# Autodesk Inventor assembly: Wheel Insert Inner Context
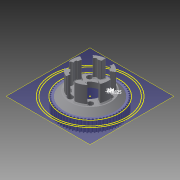
[picture p0: Inventor's stored thumbnail of the model, 180x180]
Saved by Autodesk Inventor 2015 SP1 (Build 190203100, 203)
## iProperties
Created: 2014-05-22
Part Number: Wheel Insert Inner Context
Document SubType Name: Assembly
Designer: dliu
Author: dliu
## Documents named in this file (3)
- C:\Users\dliu\Dropbox\dbhome\electric-longboard\dliu\Wheel Insert V3\Wheel Insert Inner V3 Context.iam
- C:\Users\dliu\Dropbox\dbhome\electric-longboard\dliu\Wheel Insert V3\Wheel Insert Sketch V3.ipt
- C:\Users\dliu\Dropbox\dbhome\electric-longboard\dliu\Wheel Insert V3\Wheel Insert Inner V3.ipt
## Components (2 placed, 2 different names)
1. Wheel Insert Sketch V3:1 — Mate:2, Mate:4, Mate:5
2. Wheel Insert Inner V3:1 — Flush:3, Mate:5, Mate:6
## Relationships (5: Mate 4, Flush 1)
- Mate:2: Wheel Insert Sketch V3:1
- Mate:4: Wheel Insert Sketch V3:1
- Flush:3: Wheel Insert Inner V3:1
- Mate:5: Wheel Insert Sketch V3:1 ↔ Wheel Insert Inner V3:1
- Mate:6: Wheel Insert Inner V3:1
